# Autodesk Inventor assembly: Final Design Assembly
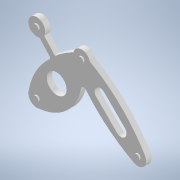
[picture p0: Inventor's stored thumbnail of the model, 180x180]
Saved by Autodesk Inventor 2021 (Build 250183000, 183)
## iProperties
Created: 2021-05-25
Part Number: Final Design Assembly
Document SubType Name: Assembly
Designer: jtri402
Author: jtri402
## Documents named in this file (3)
- \\files.auckland.ac.nz\myhome\Documents\MECHENG 334\Project B\Submission\NC Files Submission 2\Final Design Assembly.iam
- \\files.auckland.ac.nz\myhome\Documents\MECHENG 334\Project B\Submission\NC Files Submission 2\Final Bracket Design.ipt
- \\files.auckland.ac.nz\myhome\Documents\MECHENG 334\Project B\Concept Design\Pins.ipt
## Components (5 placed, 2 different names)
1. Final Bracket Design:1 — Rigid:1, Rigid:2, Rigid:3, Rigid:4
2. Pins:1 — Rigid:2
3. Pins:2 — Rigid:3
4. Pins:3 — Rigid:4
5. Pins:4 — Rigid:1
## Relationships (4: WeldJoint 4)
- Rigid:1 [WeldJoint]: Final Bracket Design:1 ↔ Pins:4
- Rigid:2 [WeldJoint]: Final Bracket Design:1 ↔ Pins:1
- Rigid:3 [WeldJoint]: Final Bracket Design:1 ↔ Pins:2
- Rigid:4 [WeldJoint]: Final Bracket Design:1 ↔ Pins:3
